# Autodesk Inventor assembly: HDR_2.54mm_RGB4078660_1
(part 3 of 3)
592. Open CASCADE STEP translator 6.8 1.452.1.592:1
593. Open CASCADE STEP translator 6.8 1.452.1.593:1
594. Open CASCADE STEP translator 6.8 1.452.1.594:1
595. Open CASCADE STEP translator 6.8 1.452.1.595:1
596. Open CASCADE STEP translator 6.8 1.452.1.596:1
597. Open CASCADE STEP translator 6.8 1.452.1.597:1
598. Open CASCADE STEP translator 6.8 1.452.1.598:1
599. Open CASCADE STEP translator 6.8 1.452.1.599:1
600. Open CASCADE STEP translator 6.8 1.452.1.600:1
601. Open CASCADE STEP translator 6.8 1.452.1.601:1
602. Open CASCADE STEP translator 6.8 1.452.1.602:1
603. Open CASCADE STEP translator 6.8 1.452.1.603:1
604. Open CASCADE STEP translator 6.8 1.452.1.604:1
605. Open CASCADE STEP translator 6.8 1.452.1.605:1
606. Open CASCADE STEP translator 6.8 1.452.1.606:1
607. Open CASCADE STEP translator 6.8 1.452.1.607:1
608. Open CASCADE STEP translator 6.8 1.452.1.608:1
609. Open CASCADE STEP translator 6.8 1.452.1.609:1
610. Open CASCADE STEP translator 6.8 1.452.1.610:1
611. Open CASCADE STEP translator 6.8 1.452.1.611:1
612. Open CASCADE STEP translator 6.8 1.452.1.612:1
613. Open CASCADE STEP translator 6.8 1.452.1.613:1
614. Open CASCADE STEP translator 6.8 1.452.1.614:1
615. Open CASCADE STEP translator 6.8 1.452.1.615:1
616. Open CASCADE STEP translator 6.8 1.452.1.616:1
617. Open CASCADE STEP translator 6.8 1.452.1.617:1
618. Open CASCADE STEP translator 6.8 1.452.1.618:1
619. Open CASCADE STEP translator 6.8 1.452.1.619:1
620. Open CASCADE STEP translator 6.8 1.452.1.620:1
621. Open CASCADE STEP translator 6.8 1.452.1.621:1
622. Open CASCADE STEP translator 6.8 1.452.1.622:1
623. Open CASCADE STEP translator 6.8 1.452.1.623:1
624. Open CASCADE STEP translator 6.8 1.452.1.624:1
